# Autodesk Inventor assembly: A2017_T5_01
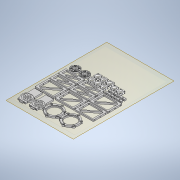
[picture p0: Inventor's stored thumbnail of the model, 180x180]
Saved by Autodesk Inventor 2020 (Build 240168000, 168)
## iProperties
Created: 2021-08-27
Part Number: A2017_T5_01
Document SubType Name: Assembly
Designer: Masato
Author: Masato
## Documents named in this file (9)
- C:\Users\naoki\Documents\Inventor\CitBrains\git_clone\OpenPlatform4_1\GFRP\OpenPlatform_ver3_0\cam\A2017_T5_01.iam
- C:\Users\naoki\Documents\Inventor\CitBrains\git_clone\OpenPlatform4_1\GFRP\OpenPlatform_ver3_0\cam\Disposable_Board.ipt
- C:\Users\naoki\Documents\Inventor\CitBrains\git_clone\OpenPlatform4_1\GFRP\OpenPlatform_ver3_0\LowerBody\Leg_joit\Leg_joint_yaw_frame.ipt
- C:\Users\naoki\Documents\Inventor\CitBrains\git_clone\OpenPlatform4_1\GFRP\OpenPlatform_ver3_0\LowerBody\Foot\Foot_root_block.ipt
- C:\Users\naoki\Documents\Inventor\CitBrains\git_clone\OpenPlatform4_1\GFRP\OpenPlatform_ver3_0\LowerBody\Link\FrontLink_diagonal.ipt
- C:\Users\naoki\Documents\Inventor\CitBrains\git_clone\OpenPlatform4_1\GFRP\OpenPlatform_ver3_0\LowerBody\Link\BackLink_diagonal.ipt
- C:\Users\naoki\Documents\Inventor\CitBrains\git_clone\OpenPlatform4_1\GFRP\OpenPlatform_ver3_0\UpperBody\Trunk\CrossRollerBearing\Outer_support_stand.ipt
- C:\Users\naoki\Documents\Inventor\CitBrains\git_clone\OpenPlatform4_1\GFRP\OpenPlatform_ver3_0\LowerBody\Knee\Knee_clamp.ipt
- C:\Users\naoki\Documents\Inventor\CitBrains\git_clone\OpenPlatform4_1\GFRP\OpenPlatform_ver3_0\UpperBody\Trunk\CrossRollerBearing\Inner_support_stand.ipt
## Components (27 placed, 8 different names)
1. Disposable_Board:1 — メイト:2, メイト:1, フラッシュ:1, フラッシュ:2, フラッシュ:3, 正接:1, 角度:1, 正接:4, フラッシュ:6, フラッシュ:8, 角度:5, 正接:11, 角度:7, 角度:8, メイト:21
2. Leg_joint_yaw_frame:1 — メイト:4, フラッシュ:3, 正接:1, フラッシュ:4, 正接:2, フラッシュ:5
3. Leg_joint_yaw_frame:2 — フラッシュ:4, 正接:2, フラッシュ:5, メイト:5, 正接:3, メイト:8
4. FrontLink_diagonal:4 — メイト:9, メイト:10, メイト:14, メイト:15
5. Outer_support_stand:1 — メイト:7, 角度:1, 正接:3, 正接:4
6. Outer_support_stand:3
7. FrontLink_diagonal:1 — メイト:6, フラッシュ:6, メイト:8, メイト:12
8. FrontLink_diagonal:2
9. FrontLink_diagonal:3 — メイト:10
10. BackLink_diagonal:1 — メイト:11, フラッシュ:8, メイト:12
11. BackLink_diagonal:3 — 正接:16
12. BackLink_diagonal:4 — メイト:14
13. BackLink_diagonal:5 — メイト:16, 正接:12, 正接:14, 正接:15
14. Foot_root_block:1 — メイト:13, メイト:15, メイト:16
15. Foot_root_block:2 — 正接:13
16. Foot_root_block:3
17. Foot_root_block:4
18. Inner_support_stand:1 — メイト:20, 角度:5, 正接:11
19. Inner_support_stand:2 — 正接:16
20. Knee_clamp:18 — 角度:7, フラッシュ:9, 正接:14
21. Knee_clamp:19
22. Knee_clamp:20
23. Knee_clamp:21
24. Knee_clamp:22 — 正接:12
25. Knee_clamp:23
26. Knee_clamp:14 — 角度:8, 正接:13, フラッシュ:9, メイト:21, 正接:15
27. Knee_clamp:24
## Component patterns: (2 elements, first: Outer_support_stand:1), (3 elements, first: FrontLink_diagonal:1), (4 elements, first: BackLink_diagonal:1), (4 elements, first: Foot_root_block:1), (2 elements, first: Inner_support_stand:1), (6 elements, first: Knee_clamp:18), (2 elements, first: Knee_clamp:14)
## Relationships (39: Mate 17, Tangent 10, Flush 8, Angle 4)
- メイト:2 [Mate]: Disposable_Board:1
- メイト:1 [Mate]: Disposable_Board:1
- フラッシュ:1 [Flush]: Disposable_Board:1
- フラッシュ:2 [Flush]: Disposable_Board:1
- メイト:4 [Mate]: Leg_joint_yaw_frame:1
- フラッシュ:3 [Flush] (3 mm): Disposable_Board:1 ↔ Leg_joint_yaw_frame:1
- 正接:1 [Tangent] (3 mm): Disposable_Board:1 ↔ Leg_joint_yaw_frame:1
- フラッシュ:4 [Flush]: Leg_joint_yaw_frame:1 ↔ Leg_joint_yaw_frame:2
- 正接:2 [Tangent] (3 mm): Leg_joint_yaw_frame:1 ↔ Leg_joint_yaw_frame:2
- フラッシュ:5 [Flush]: Leg_joint_yaw_frame:1 ↔ Leg_joint_yaw_frame:2
- メイト:5 [Mate]: Leg_joint_yaw_frame:2
- メイト:6 [Mate]: FrontLink_diagonal:1
- メイト:7 [Mate]: Outer_support_stand:1
- 角度:1 [Angle] (0 deg): Disposable_Board:1 ↔ Outer_support_stand:1
- 正接:3 [Tangent] (3 mm): Leg_joint_yaw_frame:2 ↔ Outer_support_stand:1
- 正接:4 [Tangent] (3 mm): Disposable_Board:1 ↔ Outer_support_stand:1
- フラッシュ:6 [Flush] (3 mm): Disposable_Board:1 ↔ FrontLink_diagonal:1
- メイト:8 [Mate] (3 mm): Leg_joint_yaw_frame:2 ↔ FrontLink_diagonal:1
- メイト:9 [Mate]: FrontLink_diagonal:4
- メイト:10 [Mate] (3 mm): FrontLink_diagonal:4 ↔ FrontLink_diagonal:3
- メイト:11 [Mate]: BackLink_diagonal:1
- フラッシュ:8 [Flush] (3 mm): Disposable_Board:1 ↔ BackLink_diagonal:1
- メイト:12 [Mate] (3 mm): FrontLink_diagonal:1 ↔ BackLink_diagonal:1
- メイト:13 [Mate]: Foot_root_block:1
- メイト:14 [Mate] (5 mm): FrontLink_diagonal:4 ↔ BackLink_diagonal:4
- メイト:15 [Mate] (3 mm): FrontLink_diagonal:4 ↔ Foot_root_block:1
- メイト:16 [Mate] (5 mm): BackLink_diagonal:5 ↔ Foot_root_block:1
- メイト:20 [Mate]: Inner_support_stand:1
- 角度:5 [Angle] (0 deg): Disposable_Board:1 ↔ Inner_support_stand:1
- 正接:11 [Tangent] (3 mm): Disposable_Board:1 ↔ Inner_support_stand:1
- 角度:7 [Angle] (45 deg): Disposable_Board:1 ↔ Knee_clamp:18
- 角度:8 [Angle] (45 deg): Disposable_Board:1 ↔ Knee_clamp:14
- 正接:12 [Tangent] (3 mm): BackLink_diagonal:5 ↔ Knee_clamp:22
- 正接:13 [Tangent] (2.5 mm): Foot_root_block:2 ↔ Knee_clamp:14
- フラッシュ:9 [Flush]: Knee_clamp:18 ↔ Knee_clamp:14
- メイト:21 [Mate]: Disposable_Board:1 ↔ Knee_clamp:14
- 正接:14 [Tangent] (3 mm): BackLink_diagonal:5 ↔ Knee_clamp:18
- 正接:15 [Tangent]: BackLink_diagonal:5 ↔ Knee_clamp:14
- 正接:16 [Tangent] (2.5 mm): BackLink_diagonal:3 ↔ Inner_support_stand:2
